# Autodesk Inventor assembly: 102
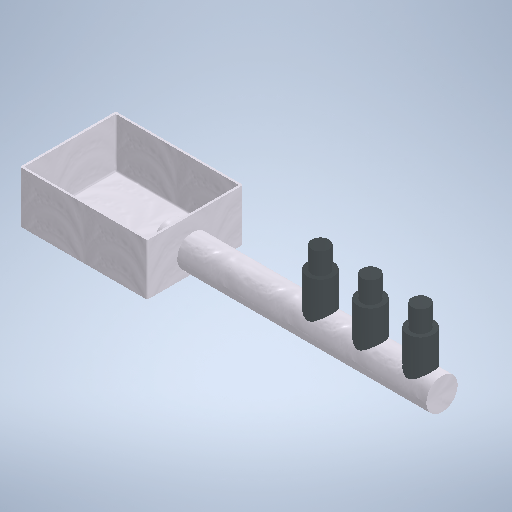
[picture p0: Inventor's stored thumbnail of the model, 512x512]
Saved by Autodesk Inventor 2025.1 (Build 291241000, 241)
## iProperties
Created: 2024-07-24
Part Number: 102
Document SubType Name: Assembly
Designer: ffogue
Author: ffogue
## Documents named in this file (4)
- C:\Projkete - Übungen\Freedom\102.iam
- C:\Projkete - Übungen\Freedom\102 part 1.ipt
- C:\Projkete - Übungen\Freedom\102 part 2.ipt
- C:\Projkete - Übungen\Freedom\102 part 3.ipt
## Components (5 placed, 3 different names)
1. 102 part 1:1 — Mate:1, Insert:1
2. 102 part 2:1 — Mate:1, Insert:1, Mate:2, Mate:3, Mate:4, Insert:2, Insert:3, Insert:4
3. 102 part 3:1 — Mate:4, Insert:4
4. 102 part 3:2 — Mate:3, Insert:3
5. 102 part 3:3 — Mate:2, Insert:2
## Relationships (8: Mate 4, Insert 4)
- Mate:1: 102 part 1:1 ↔ 102 part 2:1
- Insert:1 (-17 mm): 102 part 1:1 ↔ 102 part 2:1
- Mate:2: 102 part 2:1 ↔ 102 part 3:3
- Mate:3: 102 part 2:1 ↔ 102 part 3:2
- Mate:4: 102 part 2:1 ↔ 102 part 3:1
- Insert:2 (-11 mm): 102 part 2:1 ↔ 102 part 3:3
- Insert:3 (-11 mm): 102 part 2:1 ↔ 102 part 3:2
- Insert:4 (-11 mm): 102 part 2:1 ↔ 102 part 3:1
